# Autodesk Inventor assembly: Top_Slider Assy_3 Lanes
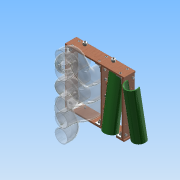
[picture p0: Inventor's stored thumbnail of the model, 180x180]
Saved by Autodesk Inventor 2018.1 (Build 221171000, 171)
## iProperties
Created: 2019-03-18
Part Number: Top_Slider Assy_3 Lanes
Document SubType Name: Assembly
Designer: James
Author: James
## Documents named in this file (23)
- C:\Users\admin\Desktop\Ball-Machine\Top Level\Top_Slider Assy_3 Lanes.iam
- C:\Users\admin\Desktop\Ball-Machine\Top Level\Top_Slider Piece 2.ipt
- C:\Users\admin\Desktop\Ball-Machine\Timing Gate\Timing_Angle Bracket.ipt
- C:\Users\admin\Desktop\Ball-Machine\Top Level\Nyloc Nut - M4.ipt
- C:\Users\admin\Desktop\Ball-Machine\Selection Sort\Socket Csk Screw - (A2) - M4 x  12.ipt
- C:\Users\admin\Desktop\Ball-Machine\Top Level\Pipes\Top_Pipe 03.ipt
- C:\Users\admin\Desktop\Ball-Machine\Top Level\Pipes\Top_Pipe 04.ipt
- C:\Users\admin\Desktop\Ball-Machine\Top Level\Pipes\Top_Pipe 05.ipt
- C:\Users\admin\Desktop\Ball-Machine\Top Level\Pipes\Top_Pipe 08.ipt
- C:\Users\admin\Desktop\Ball-Machine\Top Level\Pipes\Top_Pipe 09.ipt
- C:\Users\admin\Desktop\Ball-Machine\Top Level\Pipes\Top_Pipe 10.ipt
- C:\Users\admin\Desktop\Ball-Machine\Top Level\Socket Csk Screw - (A2) - M4 x  16.ipt
- C:\Users\admin\Desktop\Ball-Machine\Top Level\Socket Cap Screw - Standard - (A2) - M4 x 16.ipt
- C:\Users\admin\Desktop\Ball-Machine\Top Level\Top_6mm Spacer.ipt
- C:\Users\admin\Desktop\Ball-Machine\Top Level\Socket Csk Screw - (A2) - M4 x  20.ipt
- C:\Users\admin\Desktop\Ball-Machine\Top Level\Top_Slider Piece 3.ipt
- C:\Users\admin\Desktop\Ball-Machine\Top Level\Deep Groove Ball Bearing - SKF 618-6.iam
- C:\Users\admin\Desktop\Ball-Machine\Top Level\Top_Shaft 1.ipt
- C:\Users\admin\Desktop\Ball-Machine\Selection Sort\Selection_Washer.ipt
- C:\Users\admin\Desktop\Ball-Machine\Top Level\Socket Cap Screw - Standard - (A2) - M3 x 8.ipt
- C:\Users\admin\Desktop\Ball-Machine\Top Level\Socket Cap Screw - Standard - (A2) - M3 x 5.ipt
- C:\Users\admin\Desktop\Ball-Machine\Top Level\Top_Slider Piece 1_3 Lanes.ipt
- C:\Users\admin\Desktop\Ball-Machine\Top Level\Top_Tilt Pipe_3 Lanes.ipt
## Components (123 placed, 22 different names)
1. Top_Slider Piece 1_3 Lanes:1 — Mate:1, Mate:2, Flush:6, Flush:7, Mate:25, Mate:79, Mate:80, Tangent:20, Angle:8, Mate:81, Mate:82, Tangent:21, Angle:9, Mate:83, Mate:84, Tangent:22, Angle:10, Mate:85, Mate:86, Flush:26, Mate:89, Mate:90, Mate:123, Mate:134
2. Top_Slider Piece 3:1 — Flush:1, Flush:2, Flush:3, Mate:1, Flush:4, Flush:5, Flush:6, Mate:3, Mate:11, Mate:12, Mate:13, Mate:14, Mate:15, Mate:16, Mate:17, Mate:18, Mate:19, Mate:60, Mate:61, Mate:62, Mate:63, Mate:64, Tangent:2, Tangent:3, Tangent:4, Tangent:5, Tangent:10, Tangent:12, Mate:141, Mate:201, Mate:202, Mate:203, Mate:204
3. Top_Slider Piece 1_3 Lanes:2 — Flush:7, Flush:8, Mate:3, Mate:24, Mate:69, Mate:70, Mate:71, Mate:72, Mate:73, Mate:74, Tangent:14, Tangent:15, Tangent:16, Angle:3, Angle:4, Angle:5, Flush:24, Mate:91, Mate:92, Mate:124, Mate:125, Mate:129, Mate:132, Mate:135, Mate:138, Mate:139, Mate:140, Mate:148, Mate:149, Mate:150, Mate:151, Mate:161
4. Top_Slider Piece 1_3 Lanes:3 — Flush:8, Mate:126, Mate:127, Mate:128, Mate:133, Mate:136, Mate:137, Mate:141, Mate:142, Mate:143, Mate:144, Mate:145, Mate:146, Mate:147, Mate:152, Mate:153, Mate:158, Mate:160
5. Top_Slider Piece 2:2 — Mate:2, Flush:4, Flush:5, Mate:5, Mate:6, Mate:7, Flush:9, Flush:10, Mate:8, Mate:9, Mate:10, Mate:20, Mate:21, Mate:22, Mate:27, Tangent:1, Tangent:6, Tangent:7, Tangent:8, Tangent:9, Tangent:11, Mate:142, Mate:197, Mate:198, Mate:199, Mate:200
6. Top_Tilt Pipe_3 Lanes:1 — Mate:144, Mate:145, Tangent:23
7. Top_Tilt Pipe_3 Lanes:2 — Mate:139, Mate:140, Tangent:24
8. Top_6mm Spacer:1 — Mate:146, Mate:153, Tangent:23
9. Top_6mm Spacer:2 — Mate:147, Mate:152
10. Top_6mm Spacer:3 — Mate:148, Mate:150
11. Top_6mm Spacer:4 — Mate:149, Mate:151, Tangent:24
12. Socket Csk Screw - (A2) - M4 x  20:1 — Mate:164
13. Socket Csk Screw - (A2) - M4 x  20:2
14. Socket Csk Screw - (A2) - M4 x  20:3 — Mate:162
15. Socket Csk Screw - (A2) - M4 x  20:4 — Mate:163
16. Nyloc Nut - M4:46 — Mate:158
17. Nyloc Nut - M4:47 — Mate:160, Mate:163
18. Nyloc Nut - M4:48 — Flush:37, Mate:161, Mate:162
19. Nyloc Nut - M4:49 — Flush:37, Mate:164
20. Deep Groove Ball Bearing - SKF 618-6:1 [sub-assembly] — Mate:165, Mate:166
21. Top_Shaft 1:1 — Mate:165, Mate:166, Mate:167, Mate:168, Mate:171, Mate:172, Mate:198
22. Selection_Washer:1 — Mate:167, Mate:168, Mate:169, Mate:170
23. Socket Cap Screw - Standard - (A2) - M3 x 5:1 — Mate:169, Mate:170
24. Socket Cap Screw - Standard - (A2) - M3 x 8:2 — Mate:171, Mate:172, Mate:197
25. Deep Groove Ball Bearing - SKF 618-6:2 [sub-assembly]
26. Top_Shaft 1:2 — Mate:200
27. Selection_Washer:2
28. Socket Cap Screw - Standard - (A2) - M3 x 5:2
29. Socket Cap Screw - Standard - (A2) - M3 x 8:3 — Mate:199
30. Deep Groove Ball Bearing - SKF 618-6:3 [sub-assembly]
31. Top_Shaft 1:3 — Mate:204
32. Selection_Washer:3
33. Socket Cap Screw - Standard - (A2) - M3 x 5:3
34. Socket Cap Screw - Standard - (A2) - M3 x 8:4 — Mate:201
35. Deep Groove Ball Bearing - SKF 618-6:4 [sub-assembly]
36. Top_Shaft 1:4 — Mate:203
37. Selection_Washer:4
38. Socket Cap Screw - Standard - (A2) - M3 x 5:4
39. Socket Cap Screw - Standard - (A2) - M3 x 8:5 — Mate:202
40. Nyloc Nut - M4:34 — Mate:97, Mate:98
41. Socket Cap Screw - Standard - (A2) - M4 x 16:1 — Mate:97, Mate:98, Flush:27, Mate:121, Mate:123
42. Nyloc Nut - M4:35
43. Socket Cap Screw - Standard - (A2) - M4 x 16:2 — Flush:27, Mate:122
44. Nyloc Nut - M4:36
45. Socket Cap Screw - Standard - (A2) - M4 x 16:3 — Flush:28, Mate:124, Mate:138
46. Nyloc Nut - M4:37
47. Socket Cap Screw - Standard - (A2) - M4 x 16:4 — Flush:28, Mate:125
48. Nyloc Nut - M4:38
49. Socket Cap Screw - Standard - (A2) - M4 x 16:5 — Flush:29, Mate:126, Mate:137
50. Nyloc Nut - M4:39
51. Socket Cap Screw - Standard - (A2) - M4 x 16:6 — Flush:29, Mate:127
52. Nyloc Nut - M4:40
53. Socket Cap Screw - Standard - (A2) - M4 x 16:7 — Flush:30, Mate:129, Mate:135
54. Nyloc Nut - M4:41
55. Socket Cap Screw - Standard - (A2) - M4 x 16:8 — Flush:30, Mate:132
56. Nyloc Nut - M4:42
57. Socket Cap Screw - Standard - (A2) - M4 x 16:9 — Flush:31, Mate:130, Mate:134
58. Nyloc Nut - M4:43
59. Socket Cap Screw - Standard - (A2) - M4 x 16:10 — Flush:31, Mate:131
60. Nyloc Nut - M4:44
61. Socket Cap Screw - Standard - (A2) - M4 x 16:11 — Flush:32, Mate:128, Mate:136
62. Nyloc Nut - M4:45
63. Socket Cap Screw - Standard - (A2) - M4 x 16:12 — Flush:32, Mate:133
64. Timing_Angle Bracket:1 — Mate:5, Mate:6, Mate:7, Flush:9, Flush:10, Mate:25, Mate:29, Mate:54, Mate:121, Mate:122
65. Timing_Angle Bracket:2 — Mate:8, Mate:9, Mate:10, Mate:24, Mate:55, Mate:56
66. Timing_Angle Bracket:3 — Mate:11, Mate:12, Mate:13, Mate:59, Mate:130, Mate:131
67. Timing_Angle Bracket:4 — Mate:14, Mate:15, Mate:16
68. Timing_Angle Bracket:5 — Mate:20, Mate:21, Mate:22, Mate:57, Mate:58, Mate:143
69. Timing_Angle Bracket:6 — Mate:17, Mate:18, Mate:19
70. Nyloc Nut - M4:1 — Mate:28, Mate:29
71. Socket Csk Screw - (A2) - M4 x  12:1 — Mate:27, Tangent:1, Mate:28
72. Nyloc Nut - M4:2 — Flush:11, Mate:31
73. Socket Csk Screw - (A2) - M4 x  12:2 — Flush:11, Mate:31, Mate:54, Tangent:6
74. Nyloc Nut - M4:3
75. Socket Csk Screw - (A2) - M4 x  12:3 — Mate:55, Tangent:7
76. Nyloc Nut - M4:4
77. Socket Csk Screw - (A2) - M4 x  12:4 — Mate:56, Tangent:8
78. Nyloc Nut - M4:5
79. Socket Csk Screw - (A2) - M4 x  12:5 — Mate:57, Tangent:11
80. Nyloc Nut - M4:6
81. Socket Csk Screw - (A2) - M4 x  12:6 — Mate:64, Tangent:12
82. Nyloc Nut - M4:8
83. Socket Csk Screw - (A2) - M4 x  12:8 — Mate:58, Tangent:9
84. Nyloc Nut - M4:9
85. Socket Csk Screw - (A2) - M4 x  12:9 — Mate:63, Tangent:10
86. Nyloc Nut - M4:10
87. Socket Csk Screw - (A2) - M4 x  12:10 — Mate:61, Tangent:2
88. Nyloc Nut - M4:11
89. Socket Csk Screw - (A2) - M4 x  12:11 — Mate:62, Tangent:3
90. Nyloc Nut - M4:12
91. Socket Csk Screw - (A2) - M4 x  12:12 — Mate:60, Tangent:5
92. Nyloc Nut - M4:13
93. Socket Csk Screw - (A2) - M4 x  12:13 — Mate:59, Tangent:4
94. Top_Pipe 03:1 — Mate:69, Mate:70, Tangent:16, Angle:3, Mate:205, Mate:206
95. Top_Pipe 04:1 — Mate:71, Mate:72, Tangent:15, Angle:4
96. Top_Pipe 05:1 — Mate:73, Mate:74, Tangent:14, Angle:5
97. Top_Pipe 08:1 — Mate:79, Mate:80, Tangent:20, Angle:8
98. Top_Pipe 09:1 — Mate:81, Mate:82, Tangent:21, Angle:9
99. Top_Pipe 10:1 — Mate:83, Mate:84, Tangent:22, Angle:10
100. Socket Csk Screw - (A2) - M4 x  16:3 — Flush:23, Flush:24, Mate:93, Mate:205
101. Socket Csk Screw - (A2) - M4 x  16:4 — Flush:23, Mate:94, Mate:206
102. Nyloc Nut - M4:17 — Mate:92, Mate:94
103. Nyloc Nut - M4:16 — Mate:91, Mate:93
104. Socket Csk Screw - (A2) - M4 x  16:1 — Mate:85, Flush:25, Flush:26, Mate:95
105. Nyloc Nut - M4:15 — Mate:89, Mate:95
106. Socket Csk Screw - (A2) - M4 x  16:2 — Mate:86, Flush:25, Mate:96
107. Nyloc Nut - M4:14 — Mate:90, Mate:96
108. Socket Csk Screw - (A2) - M4 x  16:5
109. Socket Csk Screw - (A2) - M4 x  16:6
110. Nyloc Nut - M4:50
111. Nyloc Nut - M4:51
112. Socket Csk Screw - (A2) - M4 x  16:7
113. Nyloc Nut - M4:52
114. Socket Csk Screw - (A2) - M4 x  16:8
115. Nyloc Nut - M4:53
116. Socket Csk Screw - (A2) - M4 x  16:9
117. Socket Csk Screw - (A2) - M4 x  16:10
118. Nyloc Nut - M4:54
119. Nyloc Nut - M4:55
120. Socket Csk Screw - (A2) - M4 x  16:11
121. Nyloc Nut - M4:56
122. Socket Csk Screw - (A2) - M4 x  16:12
123. Nyloc Nut - M4:57
## Component patterns: (3 elements, first: Socket Csk Screw - (A2) - M4 x  16:3 + Socket Csk Screw - (A2) - M4 x  16:4 + Nyloc Nut - M4:17 + Nyloc Nut - M4:16 + Socket Csk Screw - (A2) - M4 x  16:1 + Nyloc Nut - M4:15 + Socket Csk Screw - (A2) - M4 x  16:2 + Nyloc Nut - M4:14)
## Relationships (253: Mate 191, Flush 36, Tangent 20, Angle 6)
- Flush:1: Top_Slider Piece 3:1
- Flush:2: Top_Slider Piece 3:1
- Flush:3: Top_Slider Piece 3:1
- Mate:1: Top_Slider Piece 1_3 Lanes:1 ↔ Top_Slider Piece 3:1
- Mate:2: Top_Slider Piece 1_3 Lanes:1 ↔ Top_Slider Piece 2:2
- Flush:4: Top_Slider Piece 3:1 ↔ Top_Slider Piece 2:2
- Flush:5: Top_Slider Piece 3:1 ↔ Top_Slider Piece 2:2
- Flush:6: Top_Slider Piece 1_3 Lanes:1 ↔ Top_Slider Piece 3:1
- Flush:7: Top_Slider Piece 1_3 Lanes:1 ↔ Top_Slider Piece 1_3 Lanes:2
- Flush:8: Top_Slider Piece 1_3 Lanes:2 ↔ Top_Slider Piece 1_3 Lanes:3
- Mate:3: Top_Slider Piece 3:1 ↔ Top_Slider Piece 1_3 Lanes:2
- Mate:5: Top_Slider Piece 2:2 ↔ Timing_Angle Bracket:1
- Mate:6: Top_Slider Piece 2:2 ↔ Timing_Angle Bracket:1
- Mate:7: Top_Slider Piece 2:2 ↔ Timing_Angle Bracket:1
- Flush:9: Top_Slider Piece 2:2 ↔ Timing_Angle Bracket:1
- Flush:10: Top_Slider Piece 2:2 ↔ Timing_Angle Bracket:1
- Mate:8: Top_Slider Piece 2:2 ↔ Timing_Angle Bracket:2
- Mate:9: Top_Slider Piece 2:2 ↔ Timing_Angle Bracket:2
- Mate:10: Top_Slider Piece 2:2 ↔ Timing_Angle Bracket:2
- Mate:11: Top_Slider Piece 3:1 ↔ Timing_Angle Bracket:3
- Mate:12: Top_Slider Piece 3:1 ↔ Timing_Angle Bracket:3
- Mate:13: Top_Slider Piece 3:1 ↔ Timing_Angle Bracket:3
- Mate:14: Top_Slider Piece 3:1 ↔ Timing_Angle Bracket:4
- Mate:15: Top_Slider Piece 3:1 ↔ Timing_Angle Bracket:4
- Mate:16: Top_Slider Piece 3:1 ↔ Timing_Angle Bracket:4
- Mate:17: Top_Slider Piece 3:1 ↔ Timing_Angle Bracket:6
- Mate:18: Top_Slider Piece 3:1 ↔ Timing_Angle Bracket:6
- Mate:19: Top_Slider Piece 3:1 ↔ Timing_Angle Bracket:6
- Mate:20: Top_Slider Piece 2:2 ↔ Timing_Angle Bracket:5
- Mate:21: Top_Slider Piece 2:2 ↔ Timing_Angle Bracket:5
- Mate:22: Top_Slider Piece 2:2 ↔ Timing_Angle Bracket:5
- Mate:24: Top_Slider Piece 1_3 Lanes:2 ↔ Timing_Angle Bracket:2
- Mate:25: Top_Slider Piece 1_3 Lanes:1 ↔ Timing_Angle Bracket:1
- Mate:27: Top_Slider Piece 2:2 ↔ Socket Csk Screw - (A2) - M4 x  12:1
- Tangent:1: Top_Slider Piece 2:2 ↔ Socket Csk Screw - (A2) - M4 x  12:1
- Mate:28: Nyloc Nut - M4:1 ↔ Socket Csk Screw - (A2) - M4 x  12:1
- Mate:29: Timing_Angle Bracket:1 ↔ Nyloc Nut - M4:1
- [Mate]: Nyloc Nut - M4:2 ↔ Socket Csk Screw - (A2) - M4 x  12:2
- Flush:11 (7.78 mm): Nyloc Nut - M4:2 ↔ Socket Csk Screw - (A2) - M4 x  12:2
- Mate:31: Nyloc Nut - M4:2 ↔ Socket Csk Screw - (A2) - M4 x  12:2
- [Mate]: Nyloc Nut - M4:3 ↔ Socket Csk Screw - (A2) - M4 x  12:3
- [Flush] (7.78 mm): Nyloc Nut - M4:3 ↔ Socket Csk Screw - (A2) - M4 x  12:3
- [Mate]: Nyloc Nut - M4:3 ↔ Socket Csk Screw - (A2) - M4 x  12:3
- [Mate]: Nyloc Nut - M4:4 ↔ Socket Csk Screw - (A2) - M4 x  12:4
- [Flush] (7.78 mm): Nyloc Nut - M4:4 ↔ Socket Csk Screw - (A2) - M4 x  12:4
- [Mate]: Nyloc Nut - M4:4 ↔ Socket Csk Screw - (A2) - M4 x  12:4
- [Mate]: Nyloc Nut - M4:5 ↔ Socket Csk Screw - (A2) - M4 x  12:5
- [Flush] (7.78 mm): Nyloc Nut - M4:5 ↔ Socket Csk Screw - (A2) - M4 x  12:5
- [Mate]: Nyloc Nut - M4:5 ↔ Socket Csk Screw - (A2) - M4 x  12:5
- [Mate]: Nyloc Nut - M4:6 ↔ Socket Csk Screw - (A2) - M4 x  12:6
- [Flush] (7.78 mm): Nyloc Nut - M4:6 ↔ Socket Csk Screw - (A2) - M4 x  12:6
- [Mate]: Nyloc Nut - M4:6 ↔ Socket Csk Screw - (A2) - M4 x  12:6
- [Mate]: Nyloc Nut - M4:8 ↔ Socket Csk Screw - (A2) - M4 x  12:8
- [Flush] (7.78 mm): Nyloc Nut - M4:8 ↔ Socket Csk Screw - (A2) - M4 x  12:8
- [Mate]: Nyloc Nut - M4:8 ↔ Socket Csk Screw - (A2) - M4 x  12:8
- [Mate]: Nyloc Nut - M4:9 ↔ Socket Csk Screw - (A2) - M4 x  12:9
- [Flush] (7.78 mm): Nyloc Nut - M4:9 ↔ Socket Csk Screw - (A2) - M4 x  12:9
- [Mate]: Nyloc Nut - M4:9 ↔ Socket Csk Screw - (A2) - M4 x  12:9
- [Mate]: Nyloc Nut - M4:10 ↔ Socket Csk Screw - (A2) - M4 x  12:10
- [Flush] (7.78 mm): Nyloc Nut - M4:10 ↔ Socket Csk Screw - (A2) - M4 x  12:10
- [Mate]: Nyloc Nut - M4:10 ↔ Socket Csk Screw - (A2) - M4 x  12:10
- [Mate]: Nyloc Nut - M4:11 ↔ Socket Csk Screw - (A2) - M4 x  12:11
- [Flush] (7.78 mm): Nyloc Nut - M4:11 ↔ Socket Csk Screw - (A2) - M4 x  12:11
- [Mate]: Nyloc Nut - M4:11 ↔ Socket Csk Screw - (A2) - M4 x  12:11
- [Mate]: Nyloc Nut - M4:12 ↔ Socket Csk Screw - (A2) - M4 x  12:12
- [Flush] (7.78 mm): Nyloc Nut - M4:12 ↔ Socket Csk Screw - (A2) - M4 x  12:12
- [Mate]: Nyloc Nut - M4:12 ↔ Socket Csk Screw - (A2) - M4 x  12:12
- [Mate]: Nyloc Nut - M4:13 ↔ Socket Csk Screw - (A2) - M4 x  12:13
- [Flush] (7.78 mm): Nyloc Nut - M4:13 ↔ Socket Csk Screw - (A2) - M4 x  12:13
- [Mate]: Nyloc Nut - M4:13 ↔ Socket Csk Screw - (A2) - M4 x  12:13
- Mate:54: Timing_Angle Bracket:1 ↔ Socket Csk Screw - (A2) - M4 x  12:2
- Mate:55: Timing_Angle Bracket:2 ↔ Socket Csk Screw - (A2) - M4 x  12:3
- Mate:56: Timing_Angle Bracket:2 ↔ Socket Csk Screw - (A2) - M4 x  12:4
- Mate:57: Timing_Angle Bracket:5 ↔ Socket Csk Screw - (A2) - M4 x  12:5
- Mate:58: Timing_Angle Bracket:5 ↔ Socket Csk Screw - (A2) - M4 x  12:8
- Mate:59: Timing_Angle Bracket:3 ↔ Socket Csk Screw - (A2) - M4 x  12:13
- Mate:60: Top_Slider Piece 3:1 ↔ Socket Csk Screw - (A2) - M4 x  12:12
- Mate:61: Top_Slider Piece 3:1 ↔ Socket Csk Screw - (A2) - M4 x  12:10
- Mate:62: Top_Slider Piece 3:1 ↔ Socket Csk Screw - (A2) - M4 x  12:11
- Mate:63: Top_Slider Piece 3:1 ↔ Socket Csk Screw - (A2) - M4 x  12:9
- Mate:64: Top_Slider Piece 3:1 ↔ Socket Csk Screw - (A2) - M4 x  12:6
- Tangent:2: Top_Slider Piece 3:1 ↔ Socket Csk Screw - (A2) - M4 x  12:10
- Tangent:3: Top_Slider Piece 3:1 ↔ Socket Csk Screw - (A2) - M4 x  12:11
- Tangent:4: Top_Slider Piece 3:1 ↔ Socket Csk Screw - (A2) - M4 x  12:13
- Tangent:5: Top_Slider Piece 3:1 ↔ Socket Csk Screw - (A2) - M4 x  12:12
- Tangent:6: Top_Slider Piece 2:2 ↔ Socket Csk Screw - (A2) - M4 x  12:2
- Tangent:7: Top_Slider Piece 2:2 ↔ Socket Csk Screw - (A2) - M4 x  12:3
- Tangent:8: Top_Slider Piece 2:2 ↔ Socket Csk Screw - (A2) - M4 x  12:4
- Tangent:9: Top_Slider Piece 2:2 ↔ Socket Csk Screw - (A2) - M4 x  12:8
- Tangent:10: Top_Slider Piece 3:1 ↔ Socket Csk Screw - (A2) - M4 x  12:9
- Tangent:11: Top_Slider Piece 2:2 ↔ Socket Csk Screw - (A2) - M4 x  12:5
- Tangent:12: Top_Slider Piece 3:1 ↔ Socket Csk Screw - (A2) - M4 x  12:6
- Mate:69: Top_Slider Piece 1_3 Lanes:2 ↔ Top_Pipe 03:1
- Mate:70: Top_Slider Piece 1_3 Lanes:2 ↔ Top_Pipe 03:1
- Mate:71: Top_Slider Piece 1_3 Lanes:2 ↔ Top_Pipe 04:1
- Mate:72: Top_Slider Piece 1_3 Lanes:2 ↔ Top_Pipe 04:1
- Mate:73: Top_Slider Piece 1_3 Lanes:2 ↔ Top_Pipe 05:1
- Mate:74: Top_Slider Piece 1_3 Lanes:2 ↔ Top_Pipe 05:1
- Tangent:14: Top_Slider Piece 1_3 Lanes:2 ↔ Top_Pipe 05:1
- Tangent:15: Top_Slider Piece 1_3 Lanes:2 ↔ Top_Pipe 04:1
- Tangent:16: Top_Slider Piece 1_3 Lanes:2 ↔ Top_Pipe 03:1
- Angle:3 (0 deg): Top_Slider Piece 1_3 Lanes:2 ↔ Top_Pipe 03:1
- Angle:4 (0 deg): Top_Slider Piece 1_3 Lanes:2 ↔ Top_Pipe 04:1
- Angle:5 (0 deg): Top_Slider Piece 1_3 Lanes:2 ↔ Top_Pipe 05:1
- Mate:79: Top_Slider Piece 1_3 Lanes:1 ↔ Top_Pipe 08:1
- Mate:80: Top_Slider Piece 1_3 Lanes:1 ↔ Top_Pipe 08:1
- Tangent:20: Top_Slider Piece 1_3 Lanes:1 ↔ Top_Pipe 08:1
- Angle:8 (0 deg): Top_Slider Piece 1_3 Lanes:1 ↔ Top_Pipe 08:1
- Mate:81: Top_Slider Piece 1_3 Lanes:1 ↔ Top_Pipe 09:1
- Mate:82: Top_Slider Piece 1_3 Lanes:1 ↔ Top_Pipe 09:1
- Tangent:21: Top_Slider Piece 1_3 Lanes:1 ↔ Top_Pipe 09:1
- Angle:9 (0 deg): Top_Slider Piece 1_3 Lanes:1 ↔ Top_Pipe 09:1
- Mate:83: Top_Slider Piece 1_3 Lanes:1 ↔ Top_Pipe 10:1
- Mate:84: Top_Slider Piece 1_3 Lanes:1 ↔ Top_Pipe 10:1
- Tangent:22: Top_Slider Piece 1_3 Lanes:1 ↔ Top_Pipe 10:1
- Angle:10 (0 deg): Top_Slider Piece 1_3 Lanes:1 ↔ Top_Pipe 10:1
- Mate:85: Top_Slider Piece 1_3 Lanes:1 ↔ Socket Csk Screw - (A2) - M4 x  16:1
- Mate:86: Top_Slider Piece 1_3 Lanes:1 ↔ Socket Csk Screw - (A2) - M4 x  16:2
- Flush:23: Socket Csk Screw - (A2) - M4 x  16:3 ↔ Socket Csk Screw - (A2) - M4 x  16:4
- Flush:24 (-5 mm): Top_Slider Piece 1_3 Lanes:2 ↔ Socket Csk Screw - (A2) - M4 x  16:3
- Flush:25: Socket Csk Screw - (A2) - M4 x  16:1 ↔ Socket Csk Screw - (A2) - M4 x  16:2
- Flush:26 (-5 mm): Top_Slider Piece 1_3 Lanes:1 ↔ Socket Csk Screw - (A2) - M4 x  16:1
- Mate:89: Top_Slider Piece 1_3 Lanes:1 ↔ Nyloc Nut - M4:15
- Mate:90: Top_Slider Piece 1_3 Lanes:1 ↔ Nyloc Nut - M4:14
- Mate:91: Top_Slider Piece 1_3 Lanes:2 ↔ Nyloc Nut - M4:16
- Mate:92: Top_Slider Piece 1_3 Lanes:2 ↔ Nyloc Nut - M4:17
- Mate:93: Socket Csk Screw - (A2) - M4 x  16:3 ↔ Nyloc Nut - M4:16
- Mate:94: Socket Csk Screw - (A2) - M4 x  16:4 ↔ Nyloc Nut - M4:17
- Mate:95: Socket Csk Screw - (A2) - M4 x  16:1 ↔ Nyloc Nut - M4:15
- Mate:96: Socket Csk Screw - (A2) - M4 x  16:2 ↔ Nyloc Nut - M4:14
- Mate:97: Nyloc Nut - M4:34 ↔ Socket Cap Screw - Standard - (A2) - M4 x 16:1
- Mate:98 (8 mm): Nyloc Nut - M4:34 ↔ Socket Cap Screw - Standard - (A2) - M4 x 16:1
- [Mate]: Nyloc Nut - M4:35 ↔ Socket Cap Screw - Standard - (A2) - M4 x 16:2
- [Mate] (8 mm): Nyloc Nut - M4:35 ↔ Socket Cap Screw - Standard - (A2) - M4 x 16:2
- [Mate]: Nyloc Nut - M4:36 ↔ Socket Cap Screw - Standard - (A2) - M4 x 16:3
- [Mate] (8 mm): Nyloc Nut - M4:36 ↔ Socket Cap Screw - Standard - (A2) - M4 x 16:3
- [Mate]: Nyloc Nut - M4:37 ↔ Socket Cap Screw - Standard - (A2) - M4 x 16:4
- [Mate] (8 mm): Nyloc Nut - M4:37 ↔ Socket Cap Screw - Standard - (A2) - M4 x 16:4
- [Mate]: Nyloc Nut - M4:38 ↔ Socket Cap Screw - Standard - (A2) - M4 x 16:5
- [Mate] (8 mm): Nyloc Nut - M4:38 ↔ Socket Cap Screw - Standard - (A2) - M4 x 16:5
- [Mate]: Nyloc Nut - M4:39 ↔ Socket Cap Screw - Standard - (A2) - M4 x 16:6
- [Mate] (8 mm): Nyloc Nut - M4:39 ↔ Socket Cap Screw - Standard - (A2) - M4 x 16:6
- [Mate]: Nyloc Nut - M4:40 ↔ Socket Cap Screw - Standard - (A2) - M4 x 16:7
- [Mate] (8 mm): Nyloc Nut - M4:40 ↔ Socket Cap Screw - Standard - (A2) - M4 x 16:7
- [Mate]: Nyloc Nut - M4:41 ↔ Socket Cap Screw - Standard - (A2) - M4 x 16:8
- [Mate] (8 mm): Nyloc Nut - M4:41 ↔ Socket Cap Screw - Standard - (A2) - M4 x 16:8
- [Mate]: Nyloc Nut - M4:42 ↔ Socket Cap Screw - Standard - (A2) - M4 x 16:9
- [Mate] (8 mm): Nyloc Nut - M4:42 ↔ Socket Cap Screw - Standard - (A2) - M4 x 16:9
- [Mate]: Nyloc Nut - M4:43 ↔ Socket Cap Screw - Standard - (A2) - M4 x 16:10
- [Mate] (8 mm): Nyloc Nut - M4:43 ↔ Socket Cap Screw - Standard - (A2) - M4 x 16:10
- [Mate]: Nyloc Nut - M4:44 ↔ Socket Cap Screw - Standard - (A2) - M4 x 16:11
- [Mate] (8 mm): Nyloc Nut - M4:44 ↔ Socket Cap Screw - Standard - (A2) - M4 x 16:11
- [Mate]: Nyloc Nut - M4:45 ↔ Socket Cap Screw - Standard - (A2) - M4 x 16:12
- [Mate] (8 mm): Nyloc Nut - M4:45 ↔ Socket Cap Screw - Standard - (A2) - M4 x 16:12
- Flush:27: Socket Cap Screw - Standard - (A2) - M4 x 16:1 ↔ Socket Cap Screw - Standard - (A2) - M4 x 16:2
- Mate:121: Socket Cap Screw - Standard - (A2) - M4 x 16:1 ↔ Timing_Angle Bracket:1
- Mate:122: Socket Cap Screw - Standard - (A2) - M4 x 16:2 ↔ Timing_Angle Bracket:1
- Mate:123: Top_Slider Piece 1_3 Lanes:1 ↔ Socket Cap Screw - Standard - (A2) - M4 x 16:1
- Flush:28: Socket Cap Screw - Standard - (A2) - M4 x 16:3 ↔ Socket Cap Screw - Standard - (A2) - M4 x 16:4
- Flush:29: Socket Cap Screw - Standard - (A2) - M4 x 16:5 ↔ Socket Cap Screw - Standard - (A2) - M4 x 16:6
- Mate:124: Top_Slider Piece 1_3 Lanes:2 ↔ Socket Cap Screw - Standard - (A2) - M4 x 16:3
- Mate:125: Top_Slider Piece 1_3 Lanes:2 ↔ Socket Cap Screw - Standard - (A2) - M4 x 16:4
- Mate:126: Top_Slider Piece 1_3 Lanes:3 ↔ Socket Cap Screw - Standard - (A2) - M4 x 16:5
- Mate:127: Top_Slider Piece 1_3 Lanes:3 ↔ Socket Cap Screw - Standard - (A2) - M4 x 16:6
- Flush:30: Socket Cap Screw - Standard - (A2) - M4 x 16:7 ↔ Socket Cap Screw - Standard - (A2) - M4 x 16:8
- Flush:31: Socket Cap Screw - Standard - (A2) - M4 x 16:9 ↔ Socket Cap Screw - Standard - (A2) - M4 x 16:10
- Flush:32: Socket Cap Screw - Standard - (A2) - M4 x 16:11 ↔ Socket Cap Screw - Standard - (A2) - M4 x 16:12
- Mate:128: Top_Slider Piece 1_3 Lanes:3 ↔ Socket Cap Screw - Standard - (A2) - M4 x 16:11
- Mate:129: Top_Slider Piece 1_3 Lanes:2 ↔ Socket Cap Screw - Standard - (A2) - M4 x 16:7
- Mate:130: Socket Cap Screw - Standard - (A2) - M4 x 16:9 ↔ Timing_Angle Bracket:3
- Mate:131: Socket Cap Screw - Standard - (A2) - M4 x 16:10 ↔ Timing_Angle Bracket:3
- Mate:132: Top_Slider Piece 1_3 Lanes:2 ↔ Socket Cap Screw - Standard - (A2) - M4 x 16:8
- Mate:133: Top_Slider Piece 1_3 Lanes:3 ↔ Socket Cap Screw - Standard - (A2) - M4 x 16:12
- Mate:134: Top_Slider Piece 1_3 Lanes:1 ↔ Socket Cap Screw - Standard - (A2) - M4 x 16:9
- Mate:135: Top_Slider Piece 1_3 Lanes:2 ↔ Socket Cap Screw - Standard - (A2) - M4 x 16:7
- Mate:136: Top_Slider Piece 1_3 Lanes:3 ↔ Socket Cap Screw - Standard - (A2) - M4 x 16:11
- Mate:137: Top_Slider Piece 1_3 Lanes:3 ↔ Socket Cap Screw - Standard - (A2) - M4 x 16:5
- Mate:138: Top_Slider Piece 1_3 Lanes:2 ↔ Socket Cap Screw - Standard - (A2) - M4 x 16:3
- Mate:139: Top_Slider Piece 1_3 Lanes:2 ↔ Top_Tilt Pipe_3 Lanes:2
- Mate:140: Top_Slider Piece 1_3 Lanes:2 ↔ Top_Tilt Pipe_3 Lanes:2
- Mate:141: Top_Slider Piece 3:1 ↔ Top_Slider Piece 1_3 Lanes:3
- Mate:142: Top_Slider Piece 1_3 Lanes:3 ↔ Top_Slider Piece 2:2
- Mate:143: Top_Slider Piece 1_3 Lanes:3 ↔ Timing_Angle Bracket:5
- Mate:144: Top_Slider Piece 1_3 Lanes:3 ↔ Top_Tilt Pipe_3 Lanes:1
- Mate:145: Top_Slider Piece 1_3 Lanes:3 ↔ Top_Tilt Pipe_3 Lanes:1
- Mate:146: Top_Slider Piece 1_3 Lanes:3 ↔ Top_6mm Spacer:1
- Mate:147: Top_Slider Piece 1_3 Lanes:3 ↔ Top_6mm Spacer:2
- Mate:148: Top_Slider Piece 1_3 Lanes:2 ↔ Top_6mm Spacer:3
- Mate:149: Top_Slider Piece 1_3 Lanes:2 ↔ Top_6mm Spacer:4
- Mate:150: Top_Slider Piece 1_3 Lanes:2 ↔ Top_6mm Spacer:3
- Mate:151: Top_Slider Piece 1_3 Lanes:2 ↔ Top_6mm Spacer:4
- Mate:152: Top_Slider Piece 1_3 Lanes:3 ↔ Top_6mm Spacer:2
- Mate:153: Top_Slider Piece 1_3 Lanes:3 ↔ Top_6mm Spacer:1
- Tangent:23: Top_Tilt Pipe_3 Lanes:1 ↔ Top_6mm Spacer:1
- Tangent:24: Top_Tilt Pipe_3 Lanes:2 ↔ Top_6mm Spacer:4
- [Mate]: Top_Tilt Pipe_3 Lanes:1 ↔ Socket Csk Screw - (A2) - M4 x  20:4
- [Mate]: Top_Tilt Pipe_3 Lanes:2 ↔ Socket Csk Screw - (A2) - M4 x  20:3
- [Mate]: Top_Tilt Pipe_3 Lanes:1 ↔ Socket Csk Screw - (A2) - M4 x  20:2
- [Mate]: Top_Tilt Pipe_3 Lanes:2 ↔ Socket Csk Screw - (A2) - M4 x  20:1
- [Flush] (-5 mm): Top_6mm Spacer:2 ↔ Socket Csk Screw - (A2) - M4 x  20:4
- [Flush] (-5 mm): Top_6mm Spacer:3 ↔ Socket Csk Screw - (A2) - M4 x  20:3
- [Flush]: Socket Csk Screw - (A2) - M4 x  20:1 ↔ Socket Csk Screw - (A2) - M4 x  20:3
- [Flush]: Socket Csk Screw - (A2) - M4 x  20:2 ↔ Socket Csk Screw - (A2) - M4 x  20:4
- Mate:158: Top_Slider Piece 1_3 Lanes:3 ↔ Nyloc Nut - M4:46
- [Mate]: Socket Csk Screw - (A2) - M4 x  20:2 ↔ Nyloc Nut - M4:46
- Mate:160: Top_Slider Piece 1_3 Lanes:3 ↔ Nyloc Nut - M4:47
- Flush:37: Nyloc Nut - M4:48 ↔ Nyloc Nut - M4:49
- Mate:161: Top_Slider Piece 1_3 Lanes:2 ↔ Nyloc Nut - M4:48
- Mate:162: Socket Csk Screw - (A2) - M4 x  20:3 ↔ Nyloc Nut - M4:48
- Mate:163: Socket Csk Screw - (A2) - M4 x  20:4 ↔ Nyloc Nut - M4:47
- Mate:164: Socket Csk Screw - (A2) - M4 x  20:1 ↔ Nyloc Nut - M4:49
- Mate:165: Deep Groove Ball Bearing - SKF 618-6:1 ↔ Top_Shaft 1:1
- Mate:166: Deep Groove Ball Bearing - SKF 618-6:1 ↔ Top_Shaft 1:1
- Mate:167: Top_Shaft 1:1 ↔ Selection_Washer:1
- Mate:168: Top_Shaft 1:1 ↔ Selection_Washer:1
- Mate:169: Selection_Washer:1 ↔ Socket Cap Screw - Standard - (A2) - M3 x 5:1
- Mate:170: Selection_Washer:1 ↔ Socket Cap Screw - Standard - (A2) - M3 x 5:1
- Mate:171: Top_Shaft 1:1 ↔ Socket Cap Screw - Standard - (A2) - M3 x 8:2
- Mate:172 (5 mm): Top_Shaft 1:1 ↔ Socket Cap Screw - Standard - (A2) - M3 x 8:2
- [Mate]: Deep Groove Ball Bearing - SKF 618-6:2 ↔ Top_Shaft 1:2
- [Mate]: Deep Groove Ball Bearing - SKF 618-6:2 ↔ Top_Shaft 1:2
- [Mate]: Top_Shaft 1:2 ↔ Selection_Washer:2
- [Mate]: Top_Shaft 1:2 ↔ Selection_Washer:2
- [Mate]: Selection_Washer:2 ↔ Socket Cap Screw - Standard - (A2) - M3 x 5:2
- [Mate]: Selection_Washer:2 ↔ Socket Cap Screw - Standard - (A2) - M3 x 5:2
- [Mate]: Top_Shaft 1:2 ↔ Socket Cap Screw - Standard - (A2) - M3 x 8:3
- [Mate] (5 mm): Top_Shaft 1:2 ↔ Socket Cap Screw - Standard - (A2) - M3 x 8:3
- [Mate]: Deep Groove Ball Bearing - SKF 618-6:3 ↔ Top_Shaft 1:3
- [Mate]: Deep Groove Ball Bearing - SKF 618-6:3 ↔ Top_Shaft 1:3
- [Mate]: Top_Shaft 1:3 ↔ Selection_Washer:3
- [Mate]: Top_Shaft 1:3 ↔ Selection_Washer:3
- [Mate]: Selection_Washer:3 ↔ Socket Cap Screw - Standard - (A2) - M3 x 5:3
- [Mate]: Selection_Washer:3 ↔ Socket Cap Screw - Standard - (A2) - M3 x 5:3
- [Mate]: Top_Shaft 1:3 ↔ Socket Cap Screw - Standard - (A2) - M3 x 8:4
- [Mate] (5 mm): Top_Shaft 1:3 ↔ Socket Cap Screw - Standard - (A2) - M3 x 8:4
- [Mate]: Deep Groove Ball Bearing - SKF 618-6:4 ↔ Top_Shaft 1:4
- [Mate]: Deep Groove Ball Bearing - SKF 618-6:4 ↔ Top_Shaft 1:4
- [Mate]: Top_Shaft 1:4 ↔ Selection_Washer:4
- [Mate]: Top_Shaft 1:4 ↔ Selection_Washer:4
- [Mate]: Selection_Washer:4 ↔ Socket Cap Screw - Standard - (A2) - M3 x 5:4
- [Mate]: Selection_Washer:4 ↔ Socket Cap Screw - Standard - (A2) - M3 x 5:4
- [Mate]: Top_Shaft 1:4 ↔ Socket Cap Screw - Standard - (A2) - M3 x 8:5
- [Mate] (5 mm): Top_Shaft 1:4 ↔ Socket Cap Screw - Standard - (A2) - M3 x 8:5
- Mate:197: Top_Slider Piece 2:2 ↔ Socket Cap Screw - Standard - (A2) - M3 x 8:2
- Mate:198: Top_Slider Piece 2:2 ↔ Top_Shaft 1:1
- Mate:199: Top_Slider Piece 2:2 ↔ Socket Cap Screw - Standard - (A2) - M3 x 8:3
- Mate:200: Top_Slider Piece 2:2 ↔ Top_Shaft 1:2
- Mate:201: Top_Slider Piece 3:1 ↔ Socket Cap Screw - Standard - (A2) - M3 x 8:4
- Mate:202: Top_Slider Piece 3:1 ↔ Socket Cap Screw - Standard - (A2) - M3 x 8:5
- Mate:203: Top_Slider Piece 3:1 ↔ Top_Shaft 1:4
- Mate:204: Top_Slider Piece 3:1 ↔ Top_Shaft 1:3
- Mate:205: Top_Pipe 03:1 ↔ Socket Csk Screw - (A2) - M4 x  16:3
- Mate:206: Top_Pipe 03:1 ↔ Socket Csk Screw - (A2) - M4 x  16:4
## Named parameters: d41_d39 = 0 mm, d44_d41_d39 = 0 mm, d45_d42 = 7.78 mm, d46_d43 = 0 mm, d47_d41_d39 = 0 mm, d48_d42 = 7.78 mm, d49_d43 = 0 mm, d50_d41_d39 = 0 mm, d51_d42 = 7.78 mm, d52_d43 = 0 mm, d53_d41_d39 = 0 mm, d54_d42 = 7.78 mm, d55_d43 = 0 mm, d59_d41_d39 = 0 mm, d60_d42 = 7.78 mm, d61_d43 = 0 mm, d62_d41_d39 = 0 mm, d63_d42 = 7.78 mm, d64_d43 = 0 mm, d65_d41_d39 = 0 mm, d66_d42 = 7.78 mm, d67_d43 = 0 mm, d68_d41_d39 = 0 mm, d69_d42 = 7.78 mm, d70_d43 = 0 mm, d71_d41_d39 = 0 mm, d72_d42 = 7.78 mm, d73_d43 = 0 mm, d74_d41_d39 = 0 mm, d75_d42 = 7.78 mm, d76_d43 = 0 mm, d161_d159 = 0 mm, d162_d160 = 8 mm, d163_d159 = 0 mm, d164_d160 = 8 mm, d165_d159 = 0 mm, d166_d160 = 8 mm, d167_d159 = 0 mm, d168_d160 = 8 mm, d169_d159 = 0 mm, d170_d160 = 8 mm, d171_d159 = 0 mm, d172_d160 = 8 mm, d173_d159 = 0 mm, d174_d160 = 8 mm, d175_d159 = 0 mm, d176_d160 = 8 mm, d177_d159 = 0 mm, d178_d160 = 8 mm, d179_d159 = 0 mm, d180_d160 = 8 mm, d181_d159 = 0 mm, d182_d160 = 8 mm, d250_d242 = 0 mm, d251_d243 = 0 mm, d252_d244 = 0 mm, d253_d245 = 0 mm, d254_d246 = 0 mm, d255_d247 = 0 mm, d256_d248 = 0 mm, d257_d249 = 5 mm, d258_d242 = 0 mm, d259_d243 = 0 mm, d260_d244 = 0 mm, d261_d245 = 0 mm, d262_d246 = 0 mm, d263_d247 = 0 mm, d264_d248 = 0 mm, d265_d249 = 5 mm, d266_d242 = 0 mm, d267_d243 = 0 mm, d268_d244 = 0 mm, d269_d245 = 0 mm, d270_d246 = 0 mm, d271_d247 = 0 mm, d272_d248 = 0 mm, d273_d249 = 5 mm
